# Autodesk Inventor assembly: SS_5GL2_F
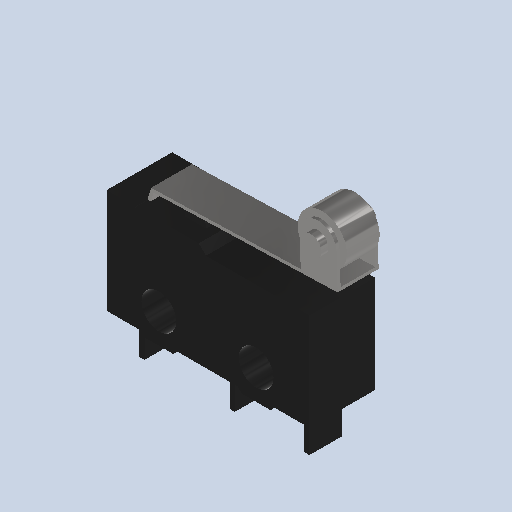
[picture p0: Inventor's stored thumbnail of the model, 512x512]
Saved by Autodesk Inventor 2022.3 (Build 263350000, 350)
## iProperties
Created: 2011-02-20
Part Number: SS_5GL2_F
Description: STEP AP203
Document SubType Name: Assembly
Designer: Hagihara Yuya
Sending System: SolidWorks 2002025
Preprocessor: SwSTEP 2.0
Title: SS_5GL2_F.step
Author: OSMC1.0
Revision Number: ANY
## Documents named in this file (3)
- C:\Users\YusukeKunita\Documents\GrabCAD\NHK2022\BasicParts\LimitSwitch\SS_5GL2_F.iam
- C:\Users\YusukeKunita\Documents\GrabCAD\NHK2022\BasicParts\LimitSwitch\SS_5GL2_F_ACTUATOR.ipt
- C:\Users\YusukeKunita\Documents\GrabCAD\NHK2022\BasicParts\LimitSwitch\SS_5GL2_F_BASE.ipt
## Components (2 placed, 2 different names)
1. SS_5GL2_F_ACTUATOR_1 — メイト:1, フラッシュ:1
2. SS_5GL2_F_BASE_2 — メイト:1, フラッシュ:1
## Relationships (2: Mate 1, Flush 1)
- メイト:1 [Mate]: SS_5GL2_F_ACTUATOR_1 ↔ SS_5GL2_F_BASE_2
- フラッシュ:1 [Flush] (1.2 mm): SS_5GL2_F_ACTUATOR_1 ↔ SS_5GL2_F_BASE_2
